# Autodesk Inventor assembly: DGB_000_DriveGearBox_MIR3
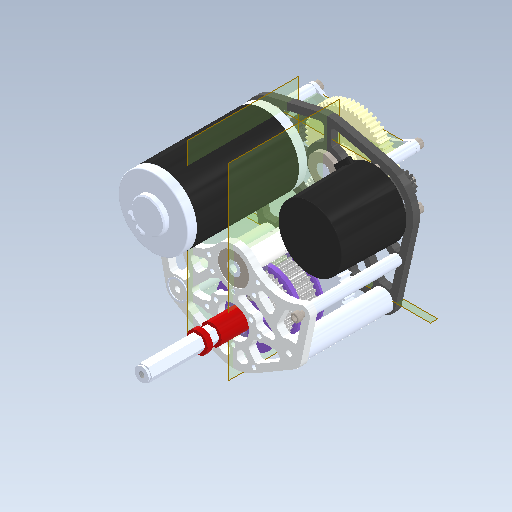
[picture p0: Inventor's stored thumbnail of the model, 512x512]
Saved by Autodesk Inventor 2020 (Build 240168000, 168)
## iProperties
Created: 2020-01-12
Part Number: DGB_000_DriveGearBox_MIR3
Document SubType Name: Assembly
Designer: turnm
Mass: 3401.94 g
Surface Area: 3275.07 cm^2
Volume: 1128.01 cm^3
Author: user
## Documents named in this file (6)
- C:\Users\turnm\Documents\GrabCAD\Infinite Recharge 2020\Build season\DGB_000_DriveGearBox_MIR3.iam
- C:\Users\turnm\Documents\GrabCAD\Infinite Recharge 2020\Build season\WCP-0155 2 Motor Flipped Gearbox_MIR2.iam
- C:\Users\turnm\Documents\GrabCAD\Infinite Recharge 2020\Build season\DGB_002_NewCover_MIR_MIR1.ipt
- C:\Users\turnm\Documents\GrabCAD\Infinite Recharge 2020\Build season\CHA_006_DrivePulleyAssembly_MIR_MIR1.iam
- C:\Users\turnm\Documents\GrabCAD\Infinite Recharge 2020\Build season\DGB_003_1.375HexSpacer_MIR_MIR1.ipt
- C:\Users\turnm\Documents\GrabCAD\Infinite Recharge 2020\Build season\DGB_004_OutputWheelSpacer_MIR_MIR1.ipt
## Components (5 placed, 5 different names)
1. WCP-0155 2 Motor Flipped Gearbox_MIR2:1 [sub-assembly] — Mate:4, Mate:5, Mate:6, Mate:7, Mate:8, Mate:9, Mate:11, Mate:12, Mate:13, Mate:14
2. DGB_002_NewCover_MIR_MIR1:1 — Mate:4, Mate:5, Mate:6
3. CHA_006_DrivePulleyAssembly_MIR_MIR1:1 [sub-assembly] — Mate:7, Mate:8, Mate:9, Mate:10
4. DGB_003_1.375HexSpacer_MIR_MIR1:1 — Mate:10, Mate:11, Mate:12, Flush:1
5. DGB_004_OutputWheelSpacer_MIR_MIR1:1 — Mate:13, Mate:14, Flush:1
## Relationships (12: Mate 11, Flush 1)
- Mate:4: WCP-0155 2 Motor Flipped Gearbox_MIR2:1 ↔ DGB_002_NewCover_MIR_MIR1:1
- Mate:5: WCP-0155 2 Motor Flipped Gearbox_MIR2:1 ↔ DGB_002_NewCover_MIR_MIR1:1
- Mate:6: WCP-0155 2 Motor Flipped Gearbox_MIR2:1 ↔ DGB_002_NewCover_MIR_MIR1:1
- Mate:7: WCP-0155 2 Motor Flipped Gearbox_MIR2:1 ↔ CHA_006_DrivePulleyAssembly_MIR_MIR1:1
- Mate:8: WCP-0155 2 Motor Flipped Gearbox_MIR2:1 ↔ CHA_006_DrivePulleyAssembly_MIR_MIR1:1
- Mate:9 (3.7846 mm): WCP-0155 2 Motor Flipped Gearbox_MIR2:1 ↔ CHA_006_DrivePulleyAssembly_MIR_MIR1:1
- Mate:10: CHA_006_DrivePulleyAssembly_MIR_MIR1:1 ↔ DGB_003_1.375HexSpacer_MIR_MIR1:1
- Mate:11: WCP-0155 2 Motor Flipped Gearbox_MIR2:1 ↔ DGB_003_1.375HexSpacer_MIR_MIR1:1
- Mate:12: WCP-0155 2 Motor Flipped Gearbox_MIR2:1 ↔ DGB_003_1.375HexSpacer_MIR_MIR1:1
- Mate:13: WCP-0155 2 Motor Flipped Gearbox_MIR2:1 ↔ DGB_004_OutputWheelSpacer_MIR_MIR1:1
- Mate:14: WCP-0155 2 Motor Flipped Gearbox_MIR2:1 ↔ DGB_004_OutputWheelSpacer_MIR_MIR1:1
- Flush:1 (12.827 mm): DGB_003_1.375HexSpacer_MIR_MIR1:1 ↔ DGB_004_OutputWheelSpacer_MIR_MIR1:1
